# Autodesk Inventor assembly: złożenie
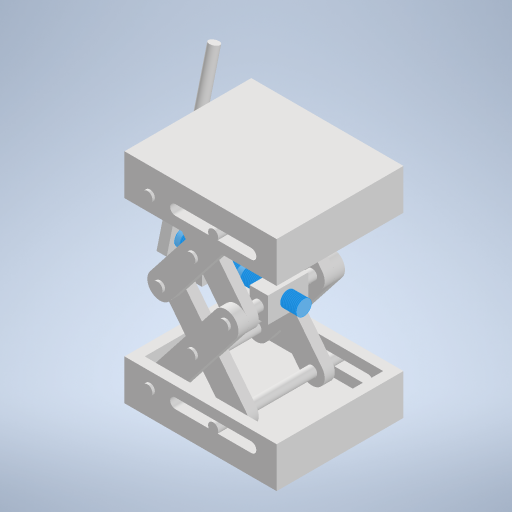
[picture p0: Inventor's stored thumbnail of the model, 512x512]
Saved by Autodesk Inventor 2024 (Build 280153000, 153)
## iProperties
Created: 2024-09-19
Part Number: złożenie
Document SubType Name: Assembly
Designer: JEDEN
Author: JEDEN
## Documents named in this file (8)
- C:\Users\JEDEN\Documents\studia\semestr 4\pp\Podstawy Konstrukcji Inżynierskich\rysunki\złożenie.iam
- C:\Users\JEDEN\Documents\studia\semestr 4\pp\Podstawy Konstrukcji Inżynierskich\rysunki\sworzeń z nakrętką.ipt
- C:\Users\JEDEN\Documents\studia\semestr 4\pp\Podstawy Konstrukcji Inżynierskich\rysunki\śruba.ipt
- C:\Users\JEDEN\Documents\studia\semestr 4\pp\Podstawy Konstrukcji Inżynierskich\rysunki\ramię.ipt
- C:\Users\JEDEN\Documents\studia\semestr 4\pp\Podstawy Konstrukcji Inżynierskich\rysunki\sworzeń1.ipt
- C:\Users\JEDEN\Documents\studia\semestr 4\pp\Podstawy Konstrukcji Inżynierskich\rysunki\sworzeń23.ipt
- C:\Users\JEDEN\Documents\studia\semestr 4\pp\Podstawy Konstrukcji Inżynierskich\rysunki\podstawa.ipt
- C:\Users\JEDEN\Documents\studia\semestr 4\pp\Podstawy Konstrukcji Inżynierskich\rysunki\dźwignia.ipt
## Components (20 placed, 7 different names)
1. sworzeń z nakrętką:1 — Obrotowe:1, Obrotowe:4, Obrotowe:9, Obrotowe:11, Walcowe:2
2. sworzeń z nakrętką:2 — Obrotowe:2, Obrotowe:3, Obrotowe:10, Obrotowe:12, Walcowe:1
3. śruba:1 — Walcowe:1, Walcowe:2, Sztywne:1
4. ramię:1 — Obrotowe:12, Obrotowe:13, Obrotowe:19
5. ramię:2 — Obrotowe:3, Obrotowe:6
6. ramię:3 — Obrotowe:11, Obrotowe:16, Obrotowe:20
7. ramię:4 — Obrotowe:10, Obrotowe:14
8. ramię:5 — Obrotowe:4, Obrotowe:5
9. ramię:6 — Obrotowe:9, Obrotowe:15
10. ramię:7 — Obrotowe:1, Obrotowe:8, Obrotowe:17
11. ramię:8 — Obrotowe:2, Obrotowe:7, Obrotowe:18
12. sworzeń1:1 — Obrotowe:18, Obrotowe:21
13. sworzeń23:1 — Obrotowe:13, Obrotowe:14, Obrotowe:15, Obrotowe:16
14. sworzeń1:2 — Obrotowe:17, przesuwne:1
15. sworzeń1:3 — Obrotowe:20, przesuwne:2
16. sworzeń1:4 — Obrotowe:19, Obrotowe:22
17. sworzeń23:5 — Obrotowe:5, Obrotowe:6, Obrotowe:7, Obrotowe:8
18. podstawa:1 — Obrotowe:21, przesuwne:1
19. podstawa:2 — Obrotowe:22, przesuwne:2
20. dźwignia:1 — Sztywne:1
## Relationships (27: RevoluteJoint 22, TranslationJoint 2, CylindricalJoint 2, WeldJoint 1)
- Obrotowe:1 [RevoluteJoint] (-5 mm): sworzeń z nakrętką:1 ↔ ramię:7
- Obrotowe:2 [RevoluteJoint] (-25 mm): sworzeń z nakrętką:2 ↔ ramię:8
- Obrotowe:3 [RevoluteJoint] (25 mm): sworzeń z nakrętką:2 ↔ ramię:2
- Obrotowe:4 [RevoluteJoint] (5 mm): sworzeń z nakrętką:1 ↔ ramię:5
- Obrotowe:5 [RevoluteJoint] (5 mm): ramię:5 ↔ sworzeń23:5
- Obrotowe:6 [RevoluteJoint] (25 mm): ramię:2 ↔ sworzeń23:5
- Obrotowe:7 [RevoluteJoint] (-25 mm): ramię:8 ↔ sworzeń23:5
- Obrotowe:8 [RevoluteJoint] (-5 mm): ramię:7 ↔ sworzeń23:5
- Obrotowe:9 [RevoluteJoint] (-25 mm): sworzeń z nakrętką:1 ↔ ramię:6
- Obrotowe:10 [RevoluteJoint] (-5 mm): sworzeń z nakrętką:2 ↔ ramię:4
- Obrotowe:11 [RevoluteJoint] (25 mm): sworzeń z nakrętką:1 ↔ ramię:3
- Obrotowe:12 [RevoluteJoint] (5 mm): sworzeń z nakrętką:2 ↔ ramię:1
- Obrotowe:13 [RevoluteJoint] (5 mm): ramię:1 ↔ sworzeń23:1
- Obrotowe:14 [RevoluteJoint] (-5 mm): ramię:4 ↔ sworzeń23:1
- Obrotowe:15 [RevoluteJoint] (-25 mm): ramię:6 ↔ sworzeń23:1
- Obrotowe:16 [RevoluteJoint] (25 mm): ramię:3 ↔ sworzeń23:1
- Obrotowe:17 [RevoluteJoint] (-25 mm): ramię:7 ↔ sworzeń1:2
- Obrotowe:18 [RevoluteJoint] (-45 mm): ramię:8 ↔ sworzeń1:1
- Obrotowe:19 [RevoluteJoint] (-25 mm): ramię:1 ↔ sworzeń1:4
- Obrotowe:20 [RevoluteJoint] (45 mm): ramię:3 ↔ sworzeń1:3
- Obrotowe:21 [RevoluteJoint] (-5 mm): sworzeń1:1 ↔ podstawa:1
- przesuwne:1 [TranslationJoint] (5 mm): sworzeń1:2 ↔ podstawa:1
- Obrotowe:22 [RevoluteJoint] (-5 mm): sworzeń1:4 ↔ podstawa:2
- przesuwne:2 [TranslationJoint] (-5 mm): sworzeń1:3 ↔ podstawa:2
- Walcowe:1 [CylindricalJoint]: sworzeń z nakrętką:2 ↔ śruba:1
- Walcowe:2 [CylindricalJoint]: sworzeń z nakrętką:1 ↔ śruba:1
- Sztywne:1 [WeldJoint]: śruba:1 ↔ dźwignia:1
